# Autodesk Inventor assembly: ASY MSC 500 BELLY
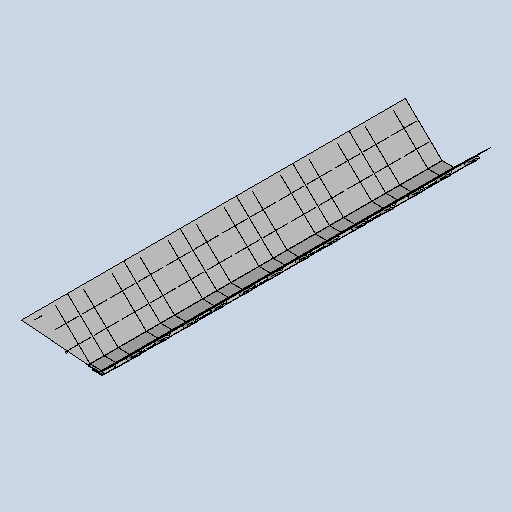
[picture p0: Inventor's stored thumbnail of the model, 512x512]
Saved by Autodesk Inventor 2025 (Build 290162010, 162A)
## iProperties
Created: 2024-07-22
Part Number: ASY MSC 500 BELLY
Document SubType Name: Assembly
Designer: pokla
Stock Number: ASY МОО 500 брюхо
Author: pokla
## Documents named in this file (6)
- C:\Users\pokla\Documents\Inventor\Отстойник осветлитель\Manturovo_Se-clar-Gleb\ASY MSC 500 BELLY.iam
- C:\Users\pokla\Documents\Inventor\Отстойник осветлитель\Manturovo_Se-clar-Gleb\MSC 501 sheet belly main.ipt
- C:\Users\pokla\Documents\Inventor\Отстойник осветлитель\Manturovo_Se-clar-Gleb\MSC 502 sheet belly-neck.ipt
- C:\Users\pokla\Documents\Inventor\Отстойник осветлитель\Manturovo_Se-clar-Gleb\MSC 504 stringer board belly.ipt
- C:\Users\pokla\Documents\Inventor\Отстойник осветлитель\Manturovo_Se-clar-Gleb\MSC 503 rib belly.ipt
- C:\Users\pokla\Documents\Inventor\Отстойник осветлитель\Manturovo_Se-clar-Gleb\MSC 505 STRINGER BOARD BELLY FACE.ipt
## Components (61 placed, 5 different names)
1. MSC 501 sheet belly main.ipt:1
2. MSC 501 sheet belly main.ipt:2
3. MSC 501 sheet belly main.ipt:3
4. MSC 502 sheet belly-neck.ipt:1 — Rigid:24
5. MSC 501 sheet belly main.ipt:4
6. MSC 501 sheet belly main.ipt:5 — Rigid:24
7. MSC 501 sheet belly main.ipt:6 — Mate:4, Mate:5, Mate:6, Mate:7, Flush:1, Mate:9, Mate:10, Flush:2, Mate:11, Mate:12
8. MSC 503 rib belly.ipt:1 — Rigid:17, Rigid:20, Rigid:21, Mate:13
9. MSC 503 rib belly.ipt:2 — Rigid:18, Rigid:19, Mate:11, Mate:12, Mate:13
10. MSC 504 stringer board belly.ipt:1 — Rigid:21, Flush:2
11. MSC 504 stringer board belly.ipt:2 — Rigid:20
12. MSC 504 stringer board belly.ipt:3 — Rigid:19
13. MSC 504 stringer board belly.ipt:4 — Rigid:18
14. MSC 506 stringer belly short.ipt:1 — Rigid:25
15. MSC 506 stringer belly short.ipt:2 — Rigid:26
16. MSC 506 stringer belly short.ipt:3 — Rigid:27
17. MSC 506 stringer belly short.ipt:4 — Rigid:28
18. MSC 504 stringer board belly.ipt:5
19. MSC 504 stringer board belly.ipt:6
20. MSC 504 stringer board belly.ipt:7
21. MSC 504 stringer board belly.ipt:8
22. MSC 504 stringer board belly.ipt:9
23. MSC 504 stringer board belly.ipt:10
24. MSC 504 stringer board belly.ipt:11
25. MSC 504 stringer board belly.ipt:12
26. MSC 504 stringer board belly.ipt:13
27. MSC 504 stringer board belly.ipt:14
28. MSC 504 stringer board belly.ipt:15
29. MSC 504 stringer board belly.ipt:16
30. MSC 504 stringer board belly.ipt:17
31. MSC 504 stringer board belly.ipt:18
32. MSC 504 stringer board belly.ipt:19
33. MSC 504 stringer board belly.ipt:20
34. MSC 504 stringer board belly.ipt:21 — Rigid:28
35. MSC 504 stringer board belly.ipt:22 — Rigid:27
36. MSC 504 stringer board belly.ipt:23 — Rigid:25
37. MSC 504 stringer board belly.ipt:24 — Rigid:26
38. MSC 503 rib belly.ipt:3 — Mate:6, Mate:7, Mate:8, Rigid:17
39. MSC 503 rib belly.ipt:4 — Mate:4, Mate:5, Mate:8
40. MSC 503 rib belly.ipt:5
41. MSC 503 rib belly.ipt:6
42. MSC 503 rib belly.ipt:7
43. MSC 503 rib belly.ipt:8
44. MSC 503 rib belly.ipt:9
45. MSC 503 rib belly.ipt:10
46. MSC 503 rib belly.ipt:11
47. MSC 503 rib belly.ipt:12
48. MSC 503 rib belly.ipt:13
49. MSC 503 rib belly.ipt:14
50. MSC 503 rib belly.ipt:15
51. MSC 503 rib belly.ipt:16
52. MSC 503 rib belly.ipt:17
53. MSC 503 rib belly.ipt:18
54. MSC 503 rib belly.ipt:19
55. MSC 503 rib belly.ipt:20
56. MSC 503 rib belly.ipt:21
57. MSC 503 rib belly.ipt:22
58. MSC 503 rib belly.ipt:23
59. MSC 503 rib belly.ipt:24
60. MSC 503 rib belly.ipt:25
61. MSC 503 rib belly.ipt:26
## Component patterns: (5 elements, first: MSC 504 stringer board belly.ipt:5 + MSC 504 stringer board belly.ipt:6 + MSC 504 stringer board belly.ipt:7 + MSC 504 stringer board belly.ipt:8), (12 elements, first: MSC 503 rib belly.ipt:3 + MSC 503 rib belly.ipt:4)
## Relationships (31: WeldJoint 19, Mate 10, Flush 2)
- [WeldJoint]: MSC 501 sheet belly main.ipt:1 ↔ MSC 501 sheet belly main.ipt:2
- [WeldJoint]: MSC 501 sheet belly main.ipt:1 ↔ MSC 501 sheet belly main.ipt:3
- [WeldJoint]: MSC 501 sheet belly main.ipt:4 ↔ MSC 501 sheet belly main.ipt:5
- [WeldJoint]: MSC 501 sheet belly main.ipt:3 ↔ MSC 501 sheet belly main.ipt:4
- [WeldJoint]: MSC 501 sheet belly main.ipt:2 ↔ MSC 501 sheet belly main.ipt:6
- [WeldJoint]: MSC 504 stringer board belly.ipt:3 ↔ MSC 504 stringer board belly.ipt:5
- [WeldJoint]: MSC 504 stringer board belly.ipt:4 ↔ MSC 504 stringer board belly.ipt:6
- [WeldJoint]: MSC 504 stringer board belly.ipt:2 ↔ MSC 504 stringer board belly.ipt:7
- [WeldJoint]: MSC 504 stringer board belly.ipt:1 ↔ MSC 504 stringer board belly.ipt:8
- Mate:4: MSC 501 sheet belly main.ipt:6 ↔ MSC 503 rib belly.ipt:4
- Mate:5: MSC 501 sheet belly main.ipt:6 ↔ MSC 503 rib belly.ipt:4
- Mate:6: MSC 501 sheet belly main.ipt:6 ↔ MSC 503 rib belly.ipt:3
- Mate:7: MSC 501 sheet belly main.ipt:6 ↔ MSC 503 rib belly.ipt:3
- Mate:8: MSC 503 rib belly.ipt:3 ↔ MSC 503 rib belly.ipt:4
- Flush:1: MSC 501 sheet belly main.ipt:6
- Mate:9: MSC 501 sheet belly main.ipt:6
- Mate:10: MSC 501 sheet belly main.ipt:6
- Rigid:17 [WeldJoint] (490 mm): MSC 503 rib belly.ipt:1 ↔ MSC 503 rib belly.ipt:3
- Rigid:18 [WeldJoint]: MSC 503 rib belly.ipt:2 ↔ MSC 504 stringer board belly.ipt:4
- Rigid:19 [WeldJoint]: MSC 503 rib belly.ipt:2 ↔ MSC 504 stringer board belly.ipt:3
- Rigid:20 [WeldJoint]: MSC 503 rib belly.ipt:1 ↔ MSC 504 stringer board belly.ipt:2
- Rigid:21 [WeldJoint]: MSC 503 rib belly.ipt:1 ↔ MSC 504 stringer board belly.ipt:1
- Flush:2: MSC 501 sheet belly main.ipt:6 ↔ MSC 504 stringer board belly.ipt:1
- Mate:11: MSC 501 sheet belly main.ipt:6 ↔ MSC 503 rib belly.ipt:2
- Mate:12: MSC 501 sheet belly main.ipt:6 ↔ MSC 503 rib belly.ipt:2
- Mate:13: MSC 503 rib belly.ipt:1 ↔ MSC 503 rib belly.ipt:2
- Rigid:24 [WeldJoint]: MSC 502 sheet belly-neck.ipt:1 ↔ MSC 501 sheet belly main.ipt:5
- Rigid:25 [WeldJoint]: MSC 506 stringer belly short.ipt:1 ↔ MSC 504 stringer board belly.ipt:23
- Rigid:26 [WeldJoint]: MSC 506 stringer belly short.ipt:2 ↔ MSC 504 stringer board belly.ipt:24
- Rigid:27 [WeldJoint]: MSC 506 stringer belly short.ipt:3 ↔ MSC 504 stringer board belly.ipt:22
- Rigid:28 [WeldJoint]: MSC 506 stringer belly short.ipt:4 ↔ MSC 504 stringer board belly.ipt:21
